# Autodesk Inventor assembly: LEG2
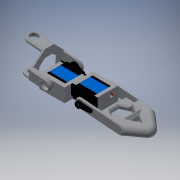
[picture p0: Inventor's stored thumbnail of the model, 180x180]
Saved by Autodesk Inventor 2017 (Build 210142000, 142)
## iProperties
Created: 2018-01-10
Part Number: LEG2
Document SubType Name: Assembly
Designer: Alex
Author: Alex
## Documents named in this file (5)
- X:\Alex\Documents\Git\HeRo-Mini\Hardware\LEG2.iam
- X:\Alex\Documents\Git\HeRo-Mini\Hardware\FEMUR.ipt
- X:\Alex\Documents\Git\HeRo-Mini\Hardware\COXA.ipt
- X:\Alex\Documents\Git\HeRo-Mini\Hardware\SERVO.iam
- X:\Alex\Documents\Git\HeRo-Mini\Hardware\TIBIA.ipt
## Components (5 placed, 4 different names)
1. FEMUR:1 — Rigid:1, Rigid:2
2. COXA:1 — Rigid:3
3. SERVO:1 [sub-assembly] — Rigid:1, Rigid:3
4. SERVO:2 [sub-assembly] — Rigid:2, Rigid:4
5. TIBIA:1 — Rigid:4
## Relationships (4: WeldJoint 4)
- Rigid:1 [WeldJoint]: FEMUR:1 ↔ SERVO:1
- Rigid:2 [WeldJoint]: FEMUR:1 ↔ SERVO:2
- Rigid:3 [WeldJoint]: COXA:1 ↔ SERVO:1
- Rigid:4 [WeldJoint]: SERVO:2 ↔ TIBIA:1
